# Autodesk Inventor assembly: RobotAsem_v3
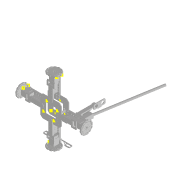
[picture p0: Inventor's stored thumbnail of the model, 180x180]
Saved by Autodesk Inventor 2022 (Build 260153000, 153)
## iProperties
Created: 2023-01-07
Part Number: RobotAsem_v3
Document SubType Name: Assembly
Designer: MVeszpremi
Author: MVeszpremi
## Documents named in this file (9)
- C:\Users\veszp\Dropbox\180DAB CAD\RobotAsem_v3.iam
- C:\Users\veszp\Dropbox\180DAB CAD\RobotBase.ipt
- C:\Users\veszp\Dropbox\180DAB CAD\SpringLoadedDesign\AssemblySpring.iam
- C:\Users\veszp\Dropbox\180DAB CAD\SpringLoadedDesign\DriverHolderInside_V2_Spring.ipt
- C:\Users\veszp\Dropbox\180DAB CAD\TrayHolder\Shaft_Mount_Lower.ipt
- C:\Users\veszp\Dropbox\180DAB CAD\TrayHolder\Shaft_2.ipt
- C:\Users\veszp\Dropbox\180DAB CAD\Vertical_Stereo_1.ipt
- C:\Users\veszp\Dropbox\180DAB CAD\Vertical_Stereo_2.ipt
- C:\Users\veszp\Dropbox\180DAB CAD\UltrasonicHolder.ipt
## Components (12 placed, 8 different names)
1. RobotBase:1 — Mate:1, Mate:2, Mate:3, Mate:4, Mate:5, Mate:6, Mate:7, Mate:8, Mate:9, Mate:10, Mate:12, Mate:16, Mate:17, Mate:18
2. RobotBase:2 — Mate:1, Mate:2, Mate:11, Mate:13, Mate:14, Mate:15
3. AssemblySpring:1 [sub-assembly] — Mate:5, Mate:6, Mate:15
4. AssemblySpring:2 [sub-assembly] — Mate:3, Mate:4, Mate:11, Mate:12
5. AssemblySpring:3 [sub-assembly] — Mate:7, Mate:8, Mate:13, Mate:30, Mate:31, Mate:32
6. AssemblySpring:4 [sub-assembly] — Mate:9, Mate:10, Mate:14, Mate:19, Mate:20, Mate:21
7. DriverHolderInside_V2_Spring:4 — Mate:16, Mate:17, Mate:18
8. Shaft_Mount_Lower:1 — Mate:19, Mate:20, Mate:21, Mate:22, Mate:23, Mate:24, Mate:25, Mate:26
9. Shaft_2:1 — Mate:22, Mate:23
10. Vertical_Stereo_1:1 — Mate:24, Mate:25, Mate:26, Mate:27, Mate:28, Mate:29
11. Vertical_Stereo_2:1 — Mate:27, Mate:28, Mate:29
12. UltrasonicHolder:1 — Mate:30, Mate:31, Mate:32
## Relationships (32: Mate 32)
- Mate:1: RobotBase:1 ↔ RobotBase:2
- Mate:2: RobotBase:1 ↔ RobotBase:2
- Mate:3: RobotBase:1 ↔ AssemblySpring:2
- Mate:4: RobotBase:1 ↔ AssemblySpring:2
- Mate:5: RobotBase:1 ↔ AssemblySpring:1
- Mate:6: RobotBase:1 ↔ AssemblySpring:1
- Mate:7: RobotBase:1 ↔ AssemblySpring:3
- Mate:8: RobotBase:1 ↔ AssemblySpring:3
- Mate:9: RobotBase:1 ↔ AssemblySpring:4
- Mate:10: RobotBase:1 ↔ AssemblySpring:4
- Mate:11 (0.05 mm): RobotBase:2 ↔ AssemblySpring:2
- Mate:12 (0.05 mm): RobotBase:1 ↔ AssemblySpring:2
- Mate:13 (0.05 mm): RobotBase:2 ↔ AssemblySpring:3
- Mate:14 (0.05 mm): RobotBase:2 ↔ AssemblySpring:4
- Mate:15 (0.05 mm): RobotBase:2 ↔ AssemblySpring:1
- Mate:16: RobotBase:1 ↔ DriverHolderInside_V2_Spring:4
- Mate:17: RobotBase:1 ↔ DriverHolderInside_V2_Spring:4
- Mate:18 (0.05 mm): RobotBase:1 ↔ DriverHolderInside_V2_Spring:4
- Mate:19: AssemblySpring:4 ↔ Shaft_Mount_Lower:1
- Mate:20: AssemblySpring:4 ↔ Shaft_Mount_Lower:1
- Mate:21: AssemblySpring:4 ↔ Shaft_Mount_Lower:1
- Mate:22: Shaft_Mount_Lower:1 ↔ Shaft_2:1
- Mate:23: Shaft_Mount_Lower:1 ↔ Shaft_2:1
- Mate:24: Shaft_Mount_Lower:1 ↔ Vertical_Stereo_1:1
- Mate:25: Shaft_Mount_Lower:1 ↔ Vertical_Stereo_1:1
- Mate:26: Shaft_Mount_Lower:1 ↔ Vertical_Stereo_1:1
- Mate:27: Vertical_Stereo_1:1 ↔ Vertical_Stereo_2:1
- Mate:28: Vertical_Stereo_1:1 ↔ Vertical_Stereo_2:1
- Mate:29: Vertical_Stereo_1:1 ↔ Vertical_Stereo_2:1
- Mate:30: AssemblySpring:3 ↔ UltrasonicHolder:1
- Mate:31: AssemblySpring:3 ↔ UltrasonicHolder:1
- Mate:32: AssemblySpring:3 ↔ UltrasonicHolder:1
